# Autodesk Inventor assembly: Maquina
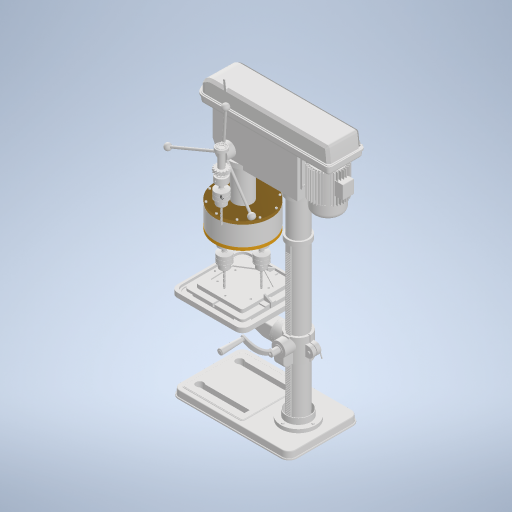
[picture p0: Inventor's stored thumbnail of the model, 512x512]
Saved by Autodesk Inventor 2024.2 (Build 282272000, 272)
## iProperties
Created: 2021-09-13
Part Number: Maquina
Description: STEP AP203
Document SubType Name: Assembly
Designer: 062210026
Sending System: SolidWorks 2018
Preprocessor: SwSTEP 2.0
Title: multi-spindle.STEP
Author: Moghimi
Revision Number: ANY
## Documents named in this file (38)
- C:\Users\062210029\Desktop\Furadeira Quase\Maquina.iam
- C:\Users\062210029\Desktop\ProjInt3\ProjInt3\Maquina\maquina\1_Varsay_lan.ipt
- C:\Users\062210029\Desktop\ProjInt3\ProjInt3\Maquina\maquina\2_Varsay_lan.ipt
- C:\Users\062210029\Desktop\ProjInt3\ProjInt3\Maquina\maquina\4_Varsay_lan.ipt
- C:\Users\062210029\Desktop\ProjInt3\ProjInt3\Maquina\maquina\5_Varsay_lan.ipt
- C:\Users\062210029\Desktop\ProjInt3\ProjInt3\Maquina\maquina\6_Varsay_lan.ipt
- C:\Users\062210029\Desktop\ProjInt3\ProjInt3\Maquina\maquina\7_Varsay_lan.ipt
- C:\Users\062210029\Desktop\ProjInt3\ProjInt3\Maquina\maquina\8_Varsay_lan.ipt
- C:\Users\062210029\Desktop\ProjInt3\ProjInt3\Maquina\maquina\9_Varsay_lan.ipt
- C:\Users\062210029\Desktop\ProjInt3\ProjInt3\Maquina\maquina\10_Varsay_lan.ipt
- C:\Users\062210029\Desktop\ProjInt3\ProjInt3\Maquina\maquina\11_Varsay_lan.ipt
- C:\Users\062210029\Desktop\ProjInt3\ProjInt3\Maquina\maquina\12_Varsay_lan.ipt
- C:\Users\062210029\Desktop\ProjInt3\ProjInt3\Maquina\maquina\13_Varsay_lan.ipt
- C:\Users\062210029\Desktop\ProjInt3\ProjInt3\Maquina\maquina\14_Varsay_lan.ipt
- C:\Users\062210029\Desktop\ProjInt3\ProjInt3\Maquina\maquina\15_Varsay_lan.ipt
- C:\Users\062210029\Desktop\ProjInt3\ProjInt3\Maquina\maquina\16_Varsay_lan.ipt
- C:\Users\062210029\Desktop\ProjInt3\ProjInt3\Maquina\maquina\hex bolt gradeab_iso_ISO 4014 - M4 x 35 x 14-N.ipt
- C:\Users\062210029\Desktop\ProjInt3\ProjInt3\Maquina\maquina\hex bolt gradeab_iso_ISO 4014 - M3 x 20 x 12-N.ipt
- C:\Users\062210029\Desktop\ProjInt3\ProjInt3\Maquina\maquina\hex bolt gradeab_iso_ISO 4014 - M6 x 30 x 18-N.ipt
- C:\Users\062210029\Desktop\ProjInt3\ProjInt3\Maquina\maquina\slotted cheese head screw_iso_ISO 1207 - M6 x 8 - 8N.ipt
- C:\Users\062210029\Desktop\ProjInt3\ProjInt3\Maquina\maquina\SKF_6004.iam
- C:\Users\062210029\Desktop\ProjInt3\ProjInt3\Maquina\maquina\MAILN AX.ipt
- C:\Users\062210029\Desktop\ProjInt3\ProjInt3\Maquina\maquina\SKF_30204.iam
- C:\Users\062210029\Desktop\ProjInt3\ProjInt3\Maquina\maquina\helical gear_3_am2_Metric - RH Helical gear 2.5M 30T 45HA 20PA 15FW ---30N75H50L35.0R1.ipt
- C:\Users\062210029\Desktop\ProjInt3\ProjInt3\Maquina\maquina\6-AX.ipt
- C:\Users\062210029\Desktop\ProjInt3\ProjInt3\Maquina\maquina\helical gear_3_am2_Metric - RH Helical gear 2.5M 15T 45HA 20PA 15FW ---15N75H50L25.0R1.ipt
- C:\Users\062210029\Desktop\ProjInt3\ProjInt3\Maquina\maquina\SHEL.ipt
- C:\Users\062210029\Desktop\ProjInt3\ProjInt3\Maquina\maquina\socket head cap screw_am_B18.3.1M - 5 x 0.8 x 20 Hex SHCS -- 20NHX.ipt
- C:\Users\062210029\Desktop\ProjInt3\ProjInt3\Maquina\maquina\STRIGHTER.ipt
- C:\Users\062210029\Desktop\ProjInt3\ProjInt3\Maquina\maquina\KEY.ipt
- C:\Users\062210029\Desktop\ProjInt3\ProjInt3\Maquina\maquina\spring pin slotted_ai_SPS 0.25x1.25.ipt
- C:\Users\062210029\Desktop\ProjInt3\ProjInt3\Maquina\maquina\socket head cap screw_am_B18.3.1M - 5 x 0.8 x 30 Hex SHCS -- 22NHX.ipt
- C:\Users\062210029\Desktop\ProjInt3\ProjInt3\Maquina\maquina\Drill.ipt
- C:\Users\062210029\Desktop\ProjInt3\ProjInt3\Maquina\maquina\FIXTURE.ipt
- C:\Users\062210029\Desktop\ProjInt3\ProjInt3\Maquina\maquina\WORKPICE.ipt
- C:\Users\062210029\Desktop\ProjInt3\ProjInt3\TampaBaixoFuras\TampaBaixo.ipt
- C:\Users\062210029\Desktop\Peças furadeira\Peças furadeira - Copia\Tampa_Superior.ipt
- C:\Users\062210029\Desktop\Ferramentas Semi Prontas\Mandril2.iam
## Components (91 placed, 79 different names)
1. Tampa_Superior:1 — Mate:12, Mate:13, Mate:14, Mate:15, Mate:16, Mate:17, Mate:18, Mate:19, Mate:20, Mate:21, Mate:22, Mate:23, Mate:24, Mate:25, Mate:26, Mate:27, Mate:28, Mate:29, Mate:30, Mate:31, Mate:32, Mate:33, Mate:34, Mate:36, Mate:37, Mate:38, Mate:39, Mate:40, Mate:41
2. Mandril2:1 [sub-assembly] — Mate:33, Mate:34
3. Mandril2:2 [sub-assembly] — Mate:36, Mate:38
4. Mandril2:4 [sub-assembly] — Mate:37, Mate:39
5. Mandril2:5 [sub-assembly] — Mate:40, Mate:41
6. SKF_30204:7 [sub-assembly]
7. helical gear_3_am2_Metric - RH Helical gear 2.5M 15T 45HA 20PA 15FW ---15N75H50L25.0R1:7
8. 6-AX:7
9. spring pin slotted_ai_SPS 0.25x1.25:7
10. 15_Varsay_lan:8
11. Drill:7
12. 1_Varsay_lan_1
13. 2_Varsay_lan_2
14. 4_Varsay_lan_3
15. 5_Varsay_lan_4
16. 6_Varsay_lan_5
17. 7_Varsay_lan_6
18. 8_Varsay_lan_7
19. 9_Varsay_lan_8
20. 10_Varsay_lan_9
21. 11_Varsay_lan_10
22. 12_Varsay_lan_11
23. 13_Varsay_lan_12
24. 14_Varsay_lan_13
25. 14_Varsay_lan_14
26. 14_Varsay_lan_15
27. 15_Varsay_lan_16
28. 16_Varsay_lan_17
29. 16_Varsay_lan_18
30. hex bolt gradeab_iso_ISO 4014 - M4 x 35 x 14-N_19
31. hex bolt gradeab_iso_ISO 4014 - M4 x 35 x 14-N_20
32. hex bolt gradeab_iso_ISO 4014 - M4 x 35 x 14-N_21
33. hex bolt gradeab_iso_ISO 4014 - M4 x 35 x 14-N_22
34. hex bolt gradeab_iso_ISO 4014 - M3 x 20 x 12-N_23
35. hex bolt gradeab_iso_ISO 4014 - M3 x 20 x 12-N_24
36. hex bolt gradeab_iso_ISO 4014 - M3 x 20 x 12-N_25
37. hex bolt gradeab_iso_ISO 4014 - M3 x 20 x 12-N_26
38. hex bolt gradeab_iso_ISO 4014 - M6 x 30 x 18-N_27
39. hex bolt gradeab_iso_ISO 4014 - M6 x 30 x 18-N_28
40. hex bolt gradeab_iso_ISO 4014 - M6 x 30 x 18-N_29
41. hex bolt gradeab_iso_ISO 4014 - M6 x 30 x 18-N_30
42. hex bolt gradeab_iso_ISO 4014 - M6 x 30 x 18-N_31
43. slotted cheese head screw_iso_ISO 1207 - M6 x 8 - 8N_32
44. SKF_6004_34 [sub-assembly]
45. SKF_6004_35 [sub-assembly] — Mate:1
46. MAILN AX_36
47. SKF_6004_39 [sub-assembly]
48. helical gear_3_am2_Metric - RH Helical gear 2.5M 30T 45HA 20PA 15FW ---30N75H50L35.0R1_40
49. SHEL_43 — Mate:12
50. socket head cap screw_am_B18.3.1M - 5 x 0.8 x 20 Hex SHCS -- 20NHX_44 — Mate:15, Mate:16
51. STRIGHTER_46
52. KEY_47
53. SKF_6004_50 [sub-assembly]
54. SKF_6004_52 [sub-assembly]
55. SKF_6004_53 [sub-assembly]
56. SKF_6004_54 [sub-assembly]
57. helical gear_3_am2_Metric - RH Helical gear 2.5M 15T 45HA 20PA 15FW ---15N75H50L25.0R1_60
58. helical gear_3_am2_Metric - RH Helical gear 2.5M 15T 45HA 20PA 15FW ---15N75H50L25.0R1_61
59. helical gear_3_am2_Metric - RH Helical gear 2.5M 15T 45HA 20PA 15FW ---15N75H50L25.0R1_62
60. helical gear_3_am2_Metric - RH Helical gear 2.5M 15T 45HA 20PA 15FW ---15N75H50L25.0R1_63
61. helical gear_3_am2_Metric - RH Helical gear 2.5M 15T 45HA 20PA 15FW ---15N75H50L25.0R1_64
62. socket head cap screw_am_B18.3.1M - 5 x 0.8 x 20 Hex SHCS -- 20NHX_70 — Mate:31, Mate:32
63. socket head cap screw_am_B18.3.1M - 5 x 0.8 x 20 Hex SHCS -- 20NHX_71 — Mate:29, Mate:30
64. socket head cap screw_am_B18.3.1M - 5 x 0.8 x 20 Hex SHCS -- 20NHX_72 — Mate:27, Mate:28
65. socket head cap screw_am_B18.3.1M - 5 x 0.8 x 20 Hex SHCS -- 20NHX_73 — Mate:25, Mate:26
66. socket head cap screw_am_B18.3.1M - 5 x 0.8 x 20 Hex SHCS -- 20NHX_75 — Mate:21, Mate:22
67. socket head cap screw_am_B18.3.1M - 5 x 0.8 x 20 Hex SHCS -- 20NHX_76 — Mate:19, Mate:20
68. socket head cap screw_am_B18.3.1M - 5 x 0.8 x 20 Hex SHCS -- 20NHX_77 — Mate:17, Mate:18
69. socket head cap screw_am_B18.3.1M - 5 x 0.8 x 20 Hex SHCS -- 20NHX_78 — Mate:13, Mate:14
70. socket head cap screw_am_B18.3.1M - 5 x 0.8 x 30 Hex SHCS -- 22NHX_98
71. socket head cap screw_am_B18.3.1M - 5 x 0.8 x 30 Hex SHCS -- 22NHX_99
72. socket head cap screw_am_B18.3.1M - 5 x 0.8 x 30 Hex SHCS -- 22NHX_100
73. socket head cap screw_am_B18.3.1M - 5 x 0.8 x 30 Hex SHCS -- 22NHX_101
74. socket head cap screw_am_B18.3.1M - 5 x 0.8 x 30 Hex SHCS -- 22NHX_102
75. socket head cap screw_am_B18.3.1M - 5 x 0.8 x 30 Hex SHCS -- 22NHX_103
76. socket head cap screw_am_B18.3.1M - 5 x 0.8 x 30 Hex SHCS -- 22NHX_104
77. FIXTURE_111
78. FIXTURE_112
79. WORKPICE_113
80. TampaBaixo:1 — Mate:1, Mate:3, Mate:4, Mate:5, Mate:6, Mate:7, Mate:8, Mate:9, Mate:10, Mate:11
81. socket head cap screw_am_B18.3.1M - 5 x 0.8 x 20 Hex SHCS -- 20NHX:21 — Mate:3
82. socket head cap screw_am_B18.3.1M - 5 x 0.8 x 20 Hex SHCS -- 20NHX:22 — Mate:8
83. socket head cap screw_am_B18.3.1M - 5 x 0.8 x 20 Hex SHCS -- 20NHX:23 — Mate:10
84. socket head cap screw_am_B18.3.1M - 5 x 0.8 x 20 Hex SHCS -- 20NHX:24
85. socket head cap screw_am_B18.3.1M - 5 x 0.8 x 20 Hex SHCS -- 20NHX:26 — Mate:5
86. socket head cap screw_am_B18.3.1M - 5 x 0.8 x 20 Hex SHCS -- 20NHX:27 — Mate:6
87. socket head cap screw_am_B18.3.1M - 5 x 0.8 x 20 Hex SHCS -- 20NHX:28 — Mate:9
88. socket head cap screw_am_B18.3.1M - 5 x 0.8 x 20 Hex SHCS -- 20NHX:30 — Mate:11
89. socket head cap screw_am_B18.3.1M - 5 x 0.8 x 20 Hex SHCS -- 20NHX:32 — Mate:7
90. socket head cap screw_am_B18.3.1M - 5 x 0.8 x 20 Hex SHCS -- 20NHX:33 — Mate:4
91. socket head cap screw_am_B18.3.1M - 5 x 0.8 x 20 Hex SHCS -- 20NHX_74 — Mate:23, Mate:24
## Relationships (39: Mate 39)
- Mate:1: SKF_6004_35 ↔ TampaBaixo:1
- Mate:3: TampaBaixo:1 ↔ socket head cap screw_am_B18.3.1M - 5 x 0.8 x 20 Hex SHCS -- 20NHX:21
- Mate:4: TampaBaixo:1 ↔ socket head cap screw_am_B18.3.1M - 5 x 0.8 x 20 Hex SHCS -- 20NHX:33
- Mate:5: TampaBaixo:1 ↔ socket head cap screw_am_B18.3.1M - 5 x 0.8 x 20 Hex SHCS -- 20NHX:26
- Mate:6: TampaBaixo:1 ↔ socket head cap screw_am_B18.3.1M - 5 x 0.8 x 20 Hex SHCS -- 20NHX:27
- Mate:7: TampaBaixo:1 ↔ socket head cap screw_am_B18.3.1M - 5 x 0.8 x 20 Hex SHCS -- 20NHX:32
- Mate:8: TampaBaixo:1 ↔ socket head cap screw_am_B18.3.1M - 5 x 0.8 x 20 Hex SHCS -- 20NHX:22
- Mate:9: TampaBaixo:1 ↔ socket head cap screw_am_B18.3.1M - 5 x 0.8 x 20 Hex SHCS -- 20NHX:28
- Mate:10: TampaBaixo:1 ↔ socket head cap screw_am_B18.3.1M - 5 x 0.8 x 20 Hex SHCS -- 20NHX:23
- Mate:11: TampaBaixo:1 ↔ socket head cap screw_am_B18.3.1M - 5 x 0.8 x 20 Hex SHCS -- 20NHX:30
- Mate:12: Tampa_Superior:1 ↔ SHEL_43
- Mate:13: Tampa_Superior:1 ↔ socket head cap screw_am_B18.3.1M - 5 x 0.8 x 20 Hex SHCS -- 20NHX_78
- Mate:14: Tampa_Superior:1 ↔ socket head cap screw_am_B18.3.1M - 5 x 0.8 x 20 Hex SHCS -- 20NHX_78
- Mate:15: Tampa_Superior:1 ↔ socket head cap screw_am_B18.3.1M - 5 x 0.8 x 20 Hex SHCS -- 20NHX_44
- Mate:16: Tampa_Superior:1 ↔ socket head cap screw_am_B18.3.1M - 5 x 0.8 x 20 Hex SHCS -- 20NHX_44
- Mate:17: Tampa_Superior:1 ↔ socket head cap screw_am_B18.3.1M - 5 x 0.8 x 20 Hex SHCS -- 20NHX_77
- Mate:18: Tampa_Superior:1 ↔ socket head cap screw_am_B18.3.1M - 5 x 0.8 x 20 Hex SHCS -- 20NHX_77
- Mate:19: Tampa_Superior:1 ↔ socket head cap screw_am_B18.3.1M - 5 x 0.8 x 20 Hex SHCS -- 20NHX_76
- Mate:20: Tampa_Superior:1 ↔ socket head cap screw_am_B18.3.1M - 5 x 0.8 x 20 Hex SHCS -- 20NHX_76
- Mate:21: Tampa_Superior:1 ↔ socket head cap screw_am_B18.3.1M - 5 x 0.8 x 20 Hex SHCS -- 20NHX_75
- Mate:22: Tampa_Superior:1 ↔ socket head cap screw_am_B18.3.1M - 5 x 0.8 x 20 Hex SHCS -- 20NHX_75
- Mate:23: Tampa_Superior:1 ↔ socket head cap screw_am_B18.3.1M - 5 x 0.8 x 20 Hex SHCS -- 20NHX_74
- Mate:24: Tampa_Superior:1 ↔ socket head cap screw_am_B18.3.1M - 5 x 0.8 x 20 Hex SHCS -- 20NHX_74
- Mate:25: Tampa_Superior:1 ↔ socket head cap screw_am_B18.3.1M - 5 x 0.8 x 20 Hex SHCS -- 20NHX_73
- Mate:26: Tampa_Superior:1 ↔ socket head cap screw_am_B18.3.1M - 5 x 0.8 x 20 Hex SHCS -- 20NHX_73
- Mate:27: Tampa_Superior:1 ↔ socket head cap screw_am_B18.3.1M - 5 x 0.8 x 20 Hex SHCS -- 20NHX_72
- Mate:28: Tampa_Superior:1 ↔ socket head cap screw_am_B18.3.1M - 5 x 0.8 x 20 Hex SHCS -- 20NHX_72
- Mate:29: Tampa_Superior:1 ↔ socket head cap screw_am_B18.3.1M - 5 x 0.8 x 20 Hex SHCS -- 20NHX_71
- Mate:30: Tampa_Superior:1 ↔ socket head cap screw_am_B18.3.1M - 5 x 0.8 x 20 Hex SHCS -- 20NHX_71
- Mate:31: Tampa_Superior:1 ↔ socket head cap screw_am_B18.3.1M - 5 x 0.8 x 20 Hex SHCS -- 20NHX_70
- Mate:32: Tampa_Superior:1 ↔ socket head cap screw_am_B18.3.1M - 5 x 0.8 x 20 Hex SHCS -- 20NHX_70
- Mate:33: Tampa_Superior:1 ↔ Mandril2:1
- Mate:34: Tampa_Superior:1 ↔ Mandril2:1
- Mate:36: Tampa_Superior:1 ↔ Mandril2:2
- Mate:37: Tampa_Superior:1 ↔ Mandril2:4
- Mate:38: Tampa_Superior:1 ↔ Mandril2:2
- Mate:39: Tampa_Superior:1 ↔ Mandril2:4
- Mate:40: Tampa_Superior:1 ↔ Mandril2:5
- Mate:41: Tampa_Superior:1 ↔ Mandril2:5
